# Autodesk Inventor assembly: atonomous_wheel_changing_robot
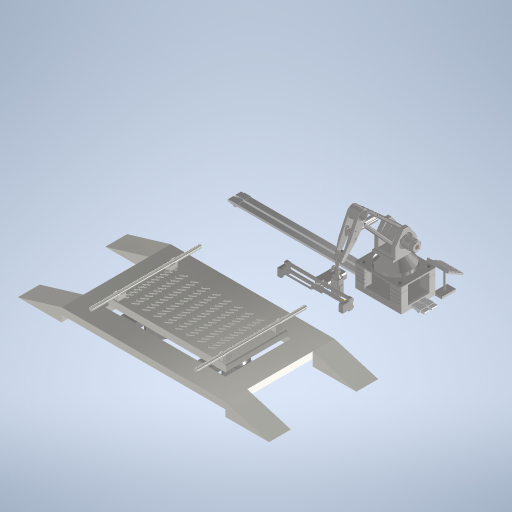
[picture p0: Inventor's stored thumbnail of the model, 512x512]
Saved by Autodesk Inventor 2023 (Build 270158000, 158)
## iProperties
Created: 2023-11-22
Part Number: atonomous_wheel_changing_robot
Document SubType Name: Assembly
Designer: Beatrice
Author: Beatrice
## Documents named in this file (3)
- E:\WORKSPACE_2\wheel_changing_assignment\atonomous_wheel_changing_robot.iam
- E:\WORKSPACE_2\wheel_changing_assignment\Complete_robotic_arm.iam
- E:\WORKSPACE_2\wheel_changing_assignment\reduced_base_platform.ipt
## Components (2 placed, 2 different names)
1. Complete_robotic_arm:1 [sub-assembly] — Flush:1, Mate:1, Flush:2
2. reduced_base_platform:1 — Flush:1, Mate:1, Flush:2
## Relationships (3: Flush 2, Mate 1)
- Flush:1: Complete_robotic_arm:1 ↔ reduced_base_platform:1
- Mate:1 (50 mm): Complete_robotic_arm:1 ↔ reduced_base_platform:1
- Flush:2: Complete_robotic_arm:1 ↔ reduced_base_platform:1
